# Autodesk Inventor assembly: Cube Line
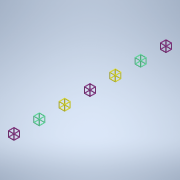
[picture p0: Inventor's stored thumbnail of the model, 180x180]
Saved by Autodesk Inventor 2021 (Build 250183000, 183)
## iProperties
Created: 2021-02-27
Part Number: Cube Line
Document SubType Name: Assembly
Designer: aidan
Author: aidan
## Documents named in this file (4)
- C:\Users\aidan\Desktop\T3 Robotics\CAD\Game Design\Cube Line.iam
- C:\Users\aidan\Desktop\T3 Robotics\CAD\Game Design\CUBE for Game Design.ipt
- C:\Users\aidan\Desktop\T3 Robotics\CAD\Game Design\CUBE for Game Design_1.ipt
- C:\Users\aidan\Desktop\T3 Robotics\CAD\Game Design\CUBE for Game Design_2.ipt
## Components (7 placed, 3 different names)
1. CUBE for Game Design:1 — Flush:1, Flush:12, Mate:1
2. CUBE for Game Design:2 — Flush:6, Flush:7, Mate:6
3. CUBE for Game Design_1:1 — Flush:1, Flush:2, Flush:11, Flush:12, Mate:1, Mate:2
4. CUBE for Game Design_1:2 — Flush:5, Flush:6, Flush:7, Flush:8, Mate:5, Mate:6
5. CUBE for Game Design_2:1 — Flush:2, Flush:3, Flush:10, Flush:11, Mate:2, Mate:3
6. CUBE for Game Design_2:2 — Flush:4, Flush:5, Flush:8, Flush:9, Mate:4, Mate:5
7. CUBE for Game Design:3 — Flush:3, Flush:4, Flush:9, Flush:10, Mate:3, Mate:4
## Relationships (18: Flush 12, Mate 6)
- Flush:1: CUBE for Game Design:1 ↔ CUBE for Game Design_1:1
- Flush:2: CUBE for Game Design_1:1 ↔ CUBE for Game Design_2:1
- Flush:3: CUBE for Game Design_2:1 ↔ CUBE for Game Design:3
- Flush:4: CUBE for Game Design_2:2 ↔ CUBE for Game Design:3
- Flush:5: CUBE for Game Design_1:2 ↔ CUBE for Game Design_2:2
- Flush:6: CUBE for Game Design:2 ↔ CUBE for Game Design_1:2
- Flush:7: CUBE for Game Design:2 ↔ CUBE for Game Design_1:2
- Flush:8: CUBE for Game Design_1:2 ↔ CUBE for Game Design_2:2
- Flush:9: CUBE for Game Design_2:2 ↔ CUBE for Game Design:3
- Flush:10: CUBE for Game Design_2:1 ↔ CUBE for Game Design:3
- Flush:11: CUBE for Game Design_1:1 ↔ CUBE for Game Design_2:1
- Flush:12: CUBE for Game Design:1 ↔ CUBE for Game Design_1:1
- Mate:1 (803.275 mm): CUBE for Game Design:1 ↔ CUBE for Game Design_1:1
- Mate:2 (803.275 mm): CUBE for Game Design_1:1 ↔ CUBE for Game Design_2:1
- Mate:3 (803.275 mm): CUBE for Game Design_2:1 ↔ CUBE for Game Design:3
- Mate:4 (803.275 mm): CUBE for Game Design_2:2 ↔ CUBE for Game Design:3
- Mate:5 (803.275 mm): CUBE for Game Design_1:2 ↔ CUBE for Game Design_2:2
- Mate:6 (803.275 mm): CUBE for Game Design:2 ↔ CUBE for Game Design_1:2
